# Autodesk Inventor assembly: Full hand
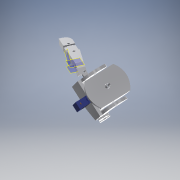
[picture p0: Inventor's stored thumbnail of the model, 180x180]
Saved by Autodesk Inventor 2018 (Build 220112000, 112)
## iProperties
Created: 2018-02-19
Part Number: Full hand
Material: Générique
Document SubType Name: Assembly
Designer: Thomas
Author: Thomas
## Documents named in this file (7)
- D:\Users\Thomas\Desktop\Projet robot augmenté\armConcept_v1\Hand\Full hand.iam
- D:\Users\Thomas\Desktop\Projet robot augmenté\armConcept_v1\Hand\Complete finger.iam
- D:\Users\Thomas\Desktop\Projet robot augmenté\armConcept_v1\Hand\Wrist.ipt
- D:\Users\Thomas\Desktop\Projet robot augmenté\armConcept_v1\Hand\palm.ipt
- D:\Users\Thomas\Desktop\Projet robot augmenté\armConcept_v1\SG90 SERVO\Micro Tower 9g v2.ipt
- D:\Users\Thomas\Desktop\Projet robot augmenté\armConcept_v1\Hand\Complete thumb.iam
- D:\Users\Thomas\Desktop\Projet robot augmenté\armConcept_v1\Hand\Hand Polley v2.ipt
## Components (9 placed, 6 different names)
1. Complete finger:1 [sub-assembly] — Rotation:3
2. Complete finger:2 [sub-assembly] — Rotation:4
3. Complete finger:3 [sub-assembly] — Rotation:6
4. Complete finger:4 [sub-assembly] — Rotation:5
5. Wrist:1 — Rotation:8
6. palm:1 — Rotation:3, Rotation:4, Rotation:5, Rotation:6, Rotation:7, Placage:1, Placage:2, Placage:3, Rotation:8
7. Micro Tower 9g v2:1 — Placage:1, Placage:2, Placage:3, Rotation:9
8. Complete thumb:1 [sub-assembly] — Rotation:7
9. Hand Polley v2:1 — Rotation:9
## Relationships (10: RevoluteJoint 7, Mate 3)
- Rotation:3 [RevoluteJoint] (-1 mm): Complete finger:1 ↔ palm:1
- Rotation:4 [RevoluteJoint] (-1 mm): Complete finger:2 ↔ palm:1
- Rotation:5 [RevoluteJoint] (-1 mm): Complete finger:4 ↔ palm:1
- Rotation:6 [RevoluteJoint] (-1 mm): Complete finger:3 ↔ palm:1
- Rotation:7 [RevoluteJoint] (-1 mm): palm:1 ↔ Complete thumb:1
- Placage:1 [Mate]: palm:1 ↔ Micro Tower 9g v2:1
- Placage:2 [Mate]: palm:1 ↔ Micro Tower 9g v2:1
- Placage:3 [Mate]: palm:1 ↔ Micro Tower 9g v2:1
- Rotation:8 [RevoluteJoint] (-2.5 mm): Wrist:1 ↔ palm:1
- Rotation:9 [RevoluteJoint]: Micro Tower 9g v2:1 ↔ Hand Polley v2:1
